# Autodesk Inventor assembly: Looks
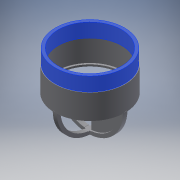
[picture p0: Inventor's stored thumbnail of the model, 180x180]
Saved by Autodesk Inventor 2016 (Build 200138000, 138)
## iProperties
Created: 2015-08-14
Part Number: Looks
Document SubType Name: Assembly
Designer: Sudhar
Author: Sudhar
## Documents named in this file (6)
- C:\Users\Sudhar\Computer Documents\Desktop\Senti-Bots\Frame Design\Version 2\Looks.iam
- C:\Users\Sudhar\Computer Documents\Desktop\Senti-Bots\Frame Design\Version 2\SentiBot top.ipt
- C:\Users\Sudhar\Computer Documents\Desktop\Senti-Bots\Frame Design\Version 2\Adapter.ipt
- C:\Users\Sudhar\Computer Documents\Desktop\Senti-Bots\Frame Design\Version 2\SentiBot botton.ipt
- C:\Users\Sudhar\Computer Documents\Desktop\Senti-Bots\Frame Design\Version 2\Control surface.ipt
- C:\Users\Sudhar\Computer Documents\Desktop\Competitions\SSC\Adapter.ipt
## Components (5 placed, 4 different names)
1. SentiBot top:1
2. Adapter:1 — Flush:1
3. SentiBot botton:1
4. Control surface:1
5. Adapter:2 — Flush:1
## Relationships (1: Flush 1)
- Flush:1: Adapter:1 ↔ Adapter:2
